# Autodesk Inventor assembly: barrel_hinge
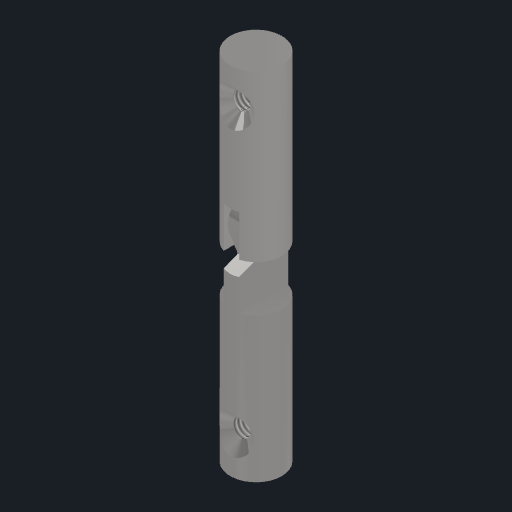
[picture p0: Inventor's stored thumbnail of the model, 512x512]
Saved by Autodesk Inventor 2023 (Build 270158000, 158)
## iProperties
Created: 2022-04-24
Part Number: barrel_hinge
Document SubType Name: Assembly
Designer: Norbert Ligas
Author: Norbert Ligas
## Documents named in this file (3)
- C:\Users\norbe\Repozytoria\NormalMapScanner\stand_construction\parts\barrel_hinge.iam
- C:\Users\norbe\Repozytoria\NormalMapScanner\stand_construction\parts\barrel_hinge-female.ipt
- C:\Users\norbe\Repozytoria\NormalMapScanner\stand_construction\parts\barrel_hinge-male.ipt
## Components (2 placed, 2 different names)
1. barrel_hinge-female:1 — Mate:1, Rotational:1
2. barrel_hinge-male:1 — Mate:1, Mate:3, Mate:4, Angle:1, Rotational:1
## Relationships (5: Mate 3, Angle 1, RevoluteJoint 1)
- Mate:1: barrel_hinge-female:1 ↔ barrel_hinge-male:1
- Mate:3: barrel_hinge-male:1
- Mate:4: barrel_hinge-male:1
- Angle:1 (0 deg): barrel_hinge-male:1
- Rotational:1 [RevoluteJoint]: barrel_hinge-female:1 ↔ barrel_hinge-male:1
